# Autodesk Inventor assembly: Assembly1
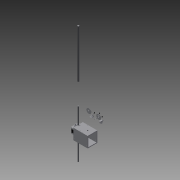
[picture p0: Inventor's stored thumbnail of the model, 180x180]
Saved by Autodesk Inventor 2015 (Build 190159000, 159)
## iProperties
Created: 2017-03-07
Part Number: Assembly1
Document SubType Name: Assembly
Designer: Ernest
Author: Ernest
## Documents named in this file (13)
- C:\Users\1esh9\Documents\Capstone-Project\doc\CAD\EndEffectorBase2\Assembly1.iam
- C:\Users\1esh9\Documents\Capstone-Project\doc\CAD\EndEffectorBase2\ThreadBar90.ipt
- C:\Users\1esh9\Documents\Capstone-Project\doc\CAD\EndEffectorBase2\ThreadBar127.ipt
- C:\Users\1esh9\Documents\Capstone-Project\doc\CAD\Stepper Motor\NEMA-17\NEMA 17.iam
- C:\Users\1esh9\Documents\Capstone-Project\doc\CAD\Gears\Spur Gears1.iam
- C:\Users\1esh9\Documents\Capstone-Project\doc\CAD\Sensors\LineSensor.ipt
- C:\Users\1esh9\Documents\Capstone-Project\doc\CAD\Sensors\LinesensorHolderBottom.ipt
- C:\Users\1esh9\Documents\Capstone-Project\doc\CAD\Sensors\LinesensorHolderTop.ipt
- C:\Users\1esh9\Documents\Capstone-Project\doc\CAD\Sensors\LinesensorHolderWasher.ipt
- C:\Users\1esh9\Documents\Capstone-Project\doc\CAD\EndEffectorBase2\BigPositionDisk.ipt
- C:\Users\1esh9\Documents\Capstone-Project\doc\CAD\EndEffectorBase2\SmallPositionDisk.ipt
- C:\Users\1esh9\Documents\Capstone-Project\doc\CAD\LowLevel_Rev3\EE_base\EE_base_assembly.iam
- C:\Users\1esh9\Documents\Capstone-Project\doc\CAD\EndEffectorBase2\BallBearing.ipt
## Components (19 placed, 12 different names)
1. ThreadBar90:1 — Mate:14, Mate:15
2. ThreadBar127:1 — Mate:15
3. NEMA 17:1 [sub-assembly] — Mate:1
4. Spur Gears:1 [sub-assembly] — Mate:1, Mate:14, Mate:16, Mate:17
5. LineSensor:1
6. LineSensor:2
7. LineSensor:3
8. LineSensor:4
9. LinesensorHolderBottom:1 — Mate:9, Mate:10, Mate:11, Mate:12, Mate:13
10. LinesensorHolderBottom:2 — Mate:5, Mate:6, Mate:7
11. LinesensorHolderTop:1 — Mate:8, Mate:12, Mate:13
12. LinesensorHolderTop:2 — Mate:2, Mate:3, Mate:4, Mate:5, Mate:7
13. LinesensorHolderWasher:1 — Mate:2, Mate:3, Mate:4, Mate:6
14. LinesensorHolderWasher:2 — Mate:8, Mate:9, Mate:10, Mate:11
15. BigPositionDisk:1
16. SmallPositionDisk:1
17. EE_base_assembly:1 [sub-assembly]
18. BallBearing:1 — Mate:16
19. BallBearing:2 — Mate:17
## Relationships (17: Mate 17)
- Mate:1: NEMA 17:1 ↔ Spur Gears:1
- Mate:2: LinesensorHolderTop:2 ↔ LinesensorHolderWasher:1
- Mate:3: LinesensorHolderTop:2 ↔ LinesensorHolderWasher:1
- Mate:4: LinesensorHolderTop:2 ↔ LinesensorHolderWasher:1
- Mate:5: LinesensorHolderBottom:2 ↔ LinesensorHolderTop:2
- Mate:6: LinesensorHolderBottom:2 ↔ LinesensorHolderWasher:1
- Mate:7: LinesensorHolderBottom:2 ↔ LinesensorHolderTop:2
- Mate:8: LinesensorHolderTop:1 ↔ LinesensorHolderWasher:2
- Mate:9: LinesensorHolderBottom:1 ↔ LinesensorHolderWasher:2
- Mate:10: LinesensorHolderBottom:1 ↔ LinesensorHolderWasher:2
- Mate:11: LinesensorHolderBottom:1 ↔ LinesensorHolderWasher:2
- Mate:12: LinesensorHolderBottom:1 ↔ LinesensorHolderTop:1
- Mate:13: LinesensorHolderBottom:1 ↔ LinesensorHolderTop:1
- Mate:14: ThreadBar90:1 ↔ Spur Gears:1
- Mate:15: ThreadBar90:1 ↔ ThreadBar127:1
- Mate:16: Spur Gears:1 ↔ BallBearing:1
- Mate:17: Spur Gears:1 ↔ BallBearing:2
